# Autodesk Inventor assembly: RobotFramewWheelAssembly
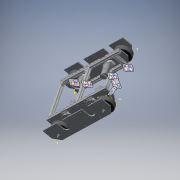
[picture p0: Inventor's stored thumbnail of the model, 180x180]
Saved by Autodesk Inventor 2016 (Build 200138000, 138)
## iProperties
Created: 2016-10-08
Part Number: RobotFramewWheelAssembly
Document SubType Name: Assembly
Designer: RoboticsUser
Author: RoboticsUser
## Documents named in this file (7)
- C:\Robotics\2016-17_CAD\RobotFramewWheelAssembly.iam
- C:\Robotics\2016-17_CAD\WheelAssemblyWFrame.iam
- C:\Robotics\CAD\2015-16\COTSParts\Bosch Extrusion\Bosch 20x20 9 in.ipt
- C:\Robotics\CAD\2015-16\COTSParts\Bosch Extrusion\Gusset 20x20 w screws.ipt
- C:\Robotics\CAD\2015-16\COTSParts\Bosch Extrusion\Bosch 20x20 9 in - Copy.ipt
- C:\Robotics\CAD\2015-16\COTSParts\Bosch Extrusion\Rexroth-6mmT-Nutm4.ipt
- C:\Robotics\CAD\2015-16\COTSParts\Bosch Extrusion\Bosch 20x20 - Copy.ipt
## Components (26 placed, 6 different names)
1. WheelAssemblyWFrame:1 [sub-assembly] — Mate:1, Insert:4, Insert:5, Insert:6
2. WheelAssemblyWFrame:2 [sub-assembly] — Mate:8, Mate:9, Flush:7, Flush:8, Insert:1, Insert:2, Insert:3
3. Bosch 20x20 9 in:1
4. Gusset 20x20 w screws:1 — Mate:9, Flush:7, Mate:10
5. Gusset 20x20 w screws:2 — Mate:1
6. Gusset 20x20 w screws:3 — Mate:8
7. Gusset 20x20 w screws:4 — Mate:11, Flush:9
8. Bosch 20x20 9 in:2 — Mate:10, Flush:8, Mate:11, Flush:9
9. Bosch 20x20 9 in - Copy:1 — Mate:33, Flush:25, Mate:38, Flush:26, Mate:43, Mate:44
10. Rexroth-6mmT-Nutm4:1 — Insert:1
11. Rexroth-6mmT-Nutm4:2 — Insert:3, Mate:33, Flush:25
12. Rexroth-6mmT-Nutm4:3 — Insert:2
13. Bosch 20x20 9 in - Copy:2 — Mate:15, Flush:11, Mate:35, Mate:39, Mate:40, Flush:27
14. Rexroth-6mmT-Nutm4:4 — Insert:4
15. Rexroth-6mmT-Nutm4:5 — Insert:5
16. Rexroth-6mmT-Nutm4:6 — Insert:6, Mate:15, Flush:11
17. Bosch 20x20 9 in:3 — Mate:41, Flush:27, Mate:42, Mate:43
18. Bosch 20x20 9 in:4 — Mate:36, Mate:37, Mate:39, Flush:26
19. Gusset 20x20 w screws:5 — Mate:37, Mate:38
20. Gusset 20x20 w screws:6 — Mate:35, Mate:36
21. Gusset 20x20 w screws:7 — Mate:40, Mate:41
22. Gusset 20x20 w screws:8 — Mate:42, Mate:44
23. Bosch 20x20 - Copy:1
24. Bosch 20x20 - Copy:2
25. Bosch 20x20 - Copy:3
26. Bosch 20x20 - Copy:4
## Relationships (30: Mate 17, Flush 7, Insert 6)
- Mate:1: WheelAssemblyWFrame:1 ↔ Gusset 20x20 w screws:2
- Mate:8: WheelAssemblyWFrame:2 ↔ Gusset 20x20 w screws:3
- Mate:9: WheelAssemblyWFrame:2 ↔ Gusset 20x20 w screws:1
- Flush:7: WheelAssemblyWFrame:2 ↔ Gusset 20x20 w screws:1
- Mate:10: Gusset 20x20 w screws:1 ↔ Bosch 20x20 9 in:2
- Flush:8: WheelAssemblyWFrame:2 ↔ Bosch 20x20 9 in:2
- Mate:11: Gusset 20x20 w screws:4 ↔ Bosch 20x20 9 in:2
- Flush:9: Gusset 20x20 w screws:4 ↔ Bosch 20x20 9 in:2
- Insert:1: WheelAssemblyWFrame:2 ↔ Rexroth-6mmT-Nutm4:1
- Insert:2: WheelAssemblyWFrame:2 ↔ Rexroth-6mmT-Nutm4:3
- Insert:3: WheelAssemblyWFrame:2 ↔ Rexroth-6mmT-Nutm4:2
- Insert:4: WheelAssemblyWFrame:1 ↔ Rexroth-6mmT-Nutm4:4
- Insert:5: WheelAssemblyWFrame:1 ↔ Rexroth-6mmT-Nutm4:5
- Insert:6: WheelAssemblyWFrame:1 ↔ Rexroth-6mmT-Nutm4:6
- Mate:15: Bosch 20x20 9 in - Copy:2 ↔ Rexroth-6mmT-Nutm4:6
- Flush:11 (64.77 mm): Bosch 20x20 9 in - Copy:2 ↔ Rexroth-6mmT-Nutm4:6
- Mate:33: Bosch 20x20 9 in - Copy:1 ↔ Rexroth-6mmT-Nutm4:2
- Flush:25 (64.77 mm): Bosch 20x20 9 in - Copy:1 ↔ Rexroth-6mmT-Nutm4:2
- Mate:35: Bosch 20x20 9 in - Copy:2 ↔ Gusset 20x20 w screws:6
- Mate:36: Bosch 20x20 9 in:4 ↔ Gusset 20x20 w screws:6
- Mate:37: Bosch 20x20 9 in:4 ↔ Gusset 20x20 w screws:5
- Mate:38: Bosch 20x20 9 in - Copy:1 ↔ Gusset 20x20 w screws:5
- Mate:39: Bosch 20x20 9 in - Copy:2 ↔ Bosch 20x20 9 in:4
- Flush:26: Bosch 20x20 9 in - Copy:1 ↔ Bosch 20x20 9 in:4
- Mate:40: Bosch 20x20 9 in - Copy:2 ↔ Gusset 20x20 w screws:7
- Mate:41: Bosch 20x20 9 in:3 ↔ Gusset 20x20 w screws:7
- Flush:27: Bosch 20x20 9 in - Copy:2 ↔ Bosch 20x20 9 in:3
- Mate:42: Bosch 20x20 9 in:3 ↔ Gusset 20x20 w screws:8
- Mate:43: Bosch 20x20 9 in - Copy:1 ↔ Bosch 20x20 9 in:3
- Mate:44: Bosch 20x20 9 in - Copy:1 ↔ Gusset 20x20 w screws:8
